# Autodesk Inventor assembly: Body Assembly
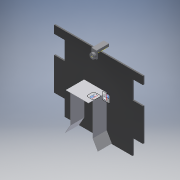
[picture p0: Inventor's stored thumbnail of the model, 180x180]
Saved by Autodesk Inventor 2019 (Build 230136000, 136)
## iProperties
Created: 2019-10-15
Part Number: Body Assembly
Document SubType Name: Assembly
Designer: User
Author: User
## Documents named in this file (5)
- C:\Robotics\CAD\2019-20_CAD\Collection\Body Assembly.iam
- C:\Robotics\CAD\2019-20_CAD\Collection\U-Part Gen 2.ipt
- C:\Robotics\CAD\COTSParts\Actobotics\545 parts\545364 assembly.ipt
- C:\Robotics\CAD\2019-20_CAD\Collection\wheel arm stand off.ipt
- C:\Robotics\CAD\2019-20_CAD\Drive Train\Gen 2.0 rev mecanums base plate.ipt
## Components (4 placed, 4 different names)
1. U-Part Gen 2:1 — Mate:19, Flush:8
2. 545364 assembly:2 — Mate:17, Mate:18
3. wheel arm stand off:2 — Mate:17, Mate:18
4. Gen 2.0 rev mecanums base plate:1 — Mate:19, Flush:8
## Relationships (4: Mate 3, Flush 1)
- Mate:17: 545364 assembly:2 ↔ wheel arm stand off:2
- Mate:18: 545364 assembly:2 ↔ wheel arm stand off:2
- Mate:19: U-Part Gen 2:1 ↔ Gen 2.0 rev mecanums base plate:1
- Flush:8 (203.2 mm): U-Part Gen 2:1 ↔ Gen 2.0 rev mecanums base plate:1
